# Autodesk Inventor assembly: Mud Kitchen 2.0
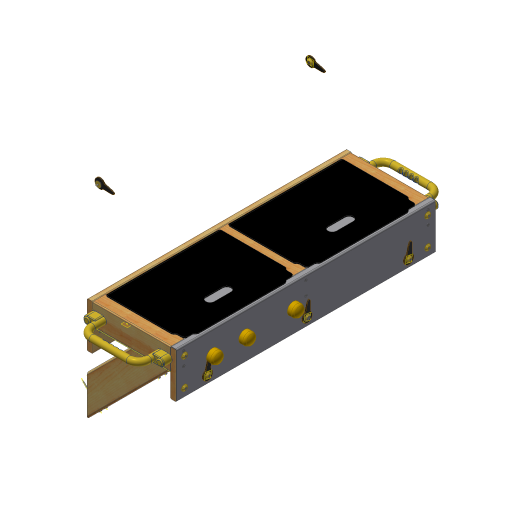
[picture p0: Inventor's stored thumbnail of the model, 512x512]
Saved by Autodesk Inventor 2024.3 (Build 283343000, 343)
## iProperties
Created: 2024-11-12
Part Number: Mud Kitchen 2.0
Document SubType Name: Assembly
Designer: l.hartouniyan
Assembly Measurements: /
Assembly Norm: /
Color: /
General Measurements: /
Packaging Manual: /
Packaging Method: /
Production Method: /
Tolerance: /
Weight: /
Author: l.hartouniyan
## Documents named in this file (14)
- Z:\Entwicklung\INVENTOR\4 Entwicklung\für 2024\24061_Mud kitchen 2.0\03_Product_development\01_3D_Construction\01_Assembly\Mud Kitchen 2.0.iam
- Z:\Entwicklung\INVENTOR\4 Entwicklung\für 2024\24061_Mud kitchen 2.0\03_Product_development\01_3D_Construction\03_Parts\Canvas\Tarp Mud Kitchen  2.0.ipt
- Z:\Entwicklung\INVENTOR\1 Teile\Holzteile\BK\Bauteile\BK-24.ipt
- Z:\Entwicklung\INVENTOR\1 Teile\Holzteile\B\Bauteile\B-80.ipt
- Z:\Entwicklung\INVENTOR\1 Teile\Holzteile\BG\Bauteile\BG-36.ipt
- Z:\Entwicklung\INVENTOR\1 Teile\Schrauben\Spannplattschrauben\Baugruppen Schrauben\5x20 inkl unterlegscheibe.iam
- Z:\Entwicklung\INVENTOR\1 Teile\Schrauben\Spannplattschrauben\Holzschraube-5x80mm.ipt
- Z:\Entwicklung\INVENTOR\1 Teile\Plastikteile\HDPE Platte\3mm\Baugruppe 3mm HDPE\Arrow Small 5x20mm washer.iam
- Z:\Entwicklung\INVENTOR\1 Teile\Schrauben\Spannplattschrauben\Holzschraube-4x50mm.ipt
- Z:\Entwicklung\INVENTOR\1 Teile\Plastikteile\GIANT\Deckel PRO gelb.ipt
- Z:\Entwicklung\INVENTOR\1 Teile\Plastikteile\GIANT\Kappe PRO gelb.ipt
- Z:\Entwicklung\INVENTOR\1 Teile\Plastikteile\Zubehör\Handgriff-gelb.ipt
- Z:\Entwicklung\INVENTOR\1 Teile\Plastikteile\Unterlegscheibe 18mm .ipt
- Z:\Entwicklung\INVENTOR\1 Teile\Plastikteile\HDPE Platte\3mm\oven deur 353 09.10 - gebogen.ipt
## Components (65 placed, 13 different names)
1. Tarp Mud Kitchen  2.0:1 — Flush:1, Flush:2, Flush:3, Flush:4, Flush:5, Flush:6, Flush:7, Mate:6, Tangent:22, Mate:7, Tangent:24, Mate:8, Tangent:26, Mate:9, Tangent:28, Mate:14, Mate:15, Tangent:57, Tangent:58, Tangent:59, Tangent:60, Mate:19, Mate:20, Mate:21, Tangent:94, Flush:56, Tangent:95, Flush:57, Mate:28
2. BK-24:1 — Flush:1, Flush:2, Flush:3, Flush:9, Mate:2, Flush:14, Mate:4, Flush:34, Tangent:49, Tangent:65, Tangent:67, Flush:46, Flush:47, Mate:18, Tangent:84, Tangent:85, Tangent:86, Tangent:87, Mate:26, Mate:30, Mate:31
3. BK-24:2 — Flush:4, Flush:5, Flush:6, Flush:8, Mate:1, Flush:10, Flush:15, Mate:5, Tangent:72, Tangent:73, Tangent:74, Tangent:75, Tangent:76, Tangent:77, Tangent:78, Tangent:79, Mate:27, Mate:33, Mate:34
4. BK-24:3 — Flush:7, Flush:8, Mate:1, Tangent:68, Tangent:69, Tangent:70, Tangent:71, Tangent:80, Tangent:81, Tangent:82, Tangent:83
5. B-80:1 — Flush:9, Flush:10, Mate:2, Tangent:21, Tangent:23, Tangent:25, Tangent:27, Tangent:50, Tangent:52, Tangent:54, Tangent:56, Flush:40, Tangent:64, Tangent:66, Tangent:88, Tangent:89, Tangent:90, Tangent:91, Tangent:92, Tangent:93
6. BG-36:1 — Flush:14, Mate:4, Tangent:45, Tangent:46, Tangent:47, Tangent:48, Tangent:51
7. BG-36:2 — Flush:15, Mate:5, Flush:30, Tangent:41, Tangent:42, Tangent:43, Tangent:44, Tangent:53, Tangent:55
8. 5x20 inkl unterlegscheibe:1 [sub-assembly] — Mate:6, Tangent:21, Tangent:22
9. 5x20 inkl unterlegscheibe:2 [sub-assembly] — Mate:7, Tangent:23, Tangent:24
10. 5x20 inkl unterlegscheibe:3 [sub-assembly] — Mate:8, Tangent:25, Tangent:26
11. 5x20 inkl unterlegscheibe:4 [sub-assembly] — Mate:9, Tangent:27, Tangent:28
12. Holzschraube-5x80mm:1 — Flush:30, Tangent:41, Tangent:42, Flush:31, Flush:32
13. Holzschraube-5x80mm:2 — Flush:31, Tangent:43, Tangent:44
14. Holzschraube-5x80mm:3 — Flush:32, Tangent:45, Tangent:46, Flush:33
15. Holzschraube-5x80mm:4 — Flush:33, Tangent:47, Tangent:48
16. Holzschraube-5x80mm:5 — Flush:34, Tangent:49, Tangent:50, Flush:35, Flush:36
17. Holzschraube-5x80mm:6 — Flush:35, Tangent:51, Tangent:52, Flush:37
18. Holzschraube-5x80mm:7 — Flush:36, Tangent:53, Tangent:54
19. Holzschraube-5x80mm:8 — Flush:37, Tangent:55, Tangent:56
20. oven deur 353 09.10 - gebogen:1 — Insert:5, Insert:6, Insert:18, Insert:19, Mate:29, Mate:30, Mate:31
21. oven deur 353 09.10 - gebogen:2 — Insert:3, Insert:4, Insert:20, Insert:21, Mate:32, Mate:33, Mate:34
22. 5x20 inkl unterlegscheibe:5 [sub-assembly] — Insert:20
23. 5x20 inkl unterlegscheibe:6 [sub-assembly] — Insert:21
24. 5x20 inkl unterlegscheibe:7 [sub-assembly] — Insert:3
25. 5x20 inkl unterlegscheibe:8 [sub-assembly] — Insert:18
26. 5x20 inkl unterlegscheibe:9 [sub-assembly] — Insert:4
27. 5x20 inkl unterlegscheibe:10 [sub-assembly] — Insert:6
28. 5x20 inkl unterlegscheibe:11 [sub-assembly] — Insert:19
29. 5x20 inkl unterlegscheibe:12 [sub-assembly] — Insert:5
30. Arrow Small 5x20mm washer:1 [sub-assembly] — Mate:15, Tangent:57, Tangent:58
31. Arrow Small 5x20mm washer:2 [sub-assembly] — Mate:14, Tangent:59, Tangent:60
32. Arrow Small 5x20mm washer:3 [sub-assembly] — Tangent:105, Flush:64, Tangent:106
33. Holzschraube-4x50mm:1 — Flush:40, Tangent:64, Tangent:65, Flush:41
34. Holzschraube-4x50mm:3 — Flush:41, Tangent:66, Tangent:67, Flush:42
35. Holzschraube-4x50mm:4 — Flush:42, Tangent:68, Tangent:69, Flush:43
36. Holzschraube-4x50mm:5 — Flush:43, Tangent:70, Tangent:71, Flush:44
37. Holzschraube-4x50mm:6 — Flush:44, Tangent:72, Tangent:73, Flush:45
38. Holzschraube-4x50mm:7 — Flush:45, Tangent:74, Tangent:75
39. B-80:2 — Flush:46, Flush:47, Mate:18, Flush:48, Flush:58, Tangent:96, Tangent:97, Flush:59, Tangent:98, Tangent:99, Flush:60, Tangent:100, Tangent:101, Flush:61, Tangent:102, Tangent:103, Tangent:105, Flush:64, Tangent:106, Flush:65, Tangent:107, Tangent:108, Mate:29, Mate:32
40. Holzschraube-4x50mm:8 — Flush:48, Tangent:76, Tangent:77, Flush:49
41. Holzschraube-4x50mm:9 — Flush:49, Tangent:78, Tangent:79, Flush:50
42. Holzschraube-4x50mm:10 — Flush:50, Tangent:80, Tangent:81, Flush:51
43. Holzschraube-4x50mm:11 — Flush:51, Tangent:82, Tangent:83, Flush:52
44. Holzschraube-4x50mm:12 — Flush:52, Tangent:84, Tangent:85, Flush:53
45. Holzschraube-4x50mm:13 — Flush:53, Tangent:86, Tangent:87
46. Deckel PRO gelb:1 — Insert:12
47. Kappe PRO gelb:1 — Tangent:88, Mate:19, Tangent:89, Insert:9, Insert:12, Insert:15
48. 5x20 inkl unterlegscheibe:13 [sub-assembly] — Insert:9
49. Kappe PRO gelb:2 — Tangent:90, Tangent:91, Mate:20, Insert:10, Insert:13, Insert:16
50. 5x20 inkl unterlegscheibe:14 [sub-assembly] — Insert:10
51. Kappe PRO gelb:3 — Tangent:92, Tangent:93, Mate:21, Insert:11, Insert:14, Insert:17
52. 5x20 inkl unterlegscheibe:15 [sub-assembly] — Insert:11
53. Deckel PRO gelb:2 — Insert:14
54. Deckel PRO gelb:3 — Insert:13
55. Arrow Small 5x20mm washer:4 [sub-assembly] — Flush:65, Tangent:107, Tangent:108
56. Handgriff-gelb:1 — Mate:26, Tangent:94, Flush:56
57. Handgriff-gelb:2 — Mate:27, Tangent:95, Flush:57
58. Holzschraube-4x50mm:14 — Flush:58, Tangent:96, Tangent:97
59. Holzschraube-4x50mm:15 — Flush:59, Tangent:98, Tangent:99
60. Holzschraube-4x50mm:16 — Flush:60, Tangent:100, Tangent:101
61. Holzschraube-4x50mm:17 — Flush:61, Tangent:102, Tangent:103
62. Unterlegscheibe 18mm :1 — Insert:15
63. Unterlegscheibe 18mm :2 — Insert:16
64. Unterlegscheibe 18mm :3 — Insert:17
65. Arrow Small 5x20mm washer:5 [sub-assembly] — Mate:28
## Relationships (154: Tangent 72, Flush 42, Mate 23, Insert 17)
- Flush:1: Tarp Mud Kitchen  2.0:1 ↔ BK-24:1
- Flush:2: Tarp Mud Kitchen  2.0:1 ↔ BK-24:1
- Flush:3: Tarp Mud Kitchen  2.0:1 ↔ BK-24:1
- Flush:4: Tarp Mud Kitchen  2.0:1 ↔ BK-24:2
- Flush:5: Tarp Mud Kitchen  2.0:1 ↔ BK-24:2
- Flush:6: Tarp Mud Kitchen  2.0:1 ↔ BK-24:2
- Flush:7: Tarp Mud Kitchen  2.0:1 ↔ BK-24:3
- Flush:8: BK-24:2 ↔ BK-24:3
- Mate:1 (334 mm): BK-24:2 ↔ BK-24:3
- Flush:9: BK-24:1 ↔ B-80:1
- Flush:10: BK-24:2 ↔ B-80:1
- Mate:2: BK-24:1 ↔ B-80:1
- Flush:14: BK-24:1 ↔ BG-36:1
- Mate:4: BK-24:1 ↔ BG-36:1
- Flush:15: BK-24:2 ↔ BG-36:2
- Mate:5: BK-24:2 ↔ BG-36:2
- Mate:6: Tarp Mud Kitchen  2.0:1 ↔ 5x20 inkl unterlegscheibe:1
- Tangent:21 (15 mm): B-80:1 ↔ 5x20 inkl unterlegscheibe:1
- Tangent:22 (15 mm): Tarp Mud Kitchen  2.0:1 ↔ 5x20 inkl unterlegscheibe:1
- Mate:7: Tarp Mud Kitchen  2.0:1 ↔ 5x20 inkl unterlegscheibe:2
- Tangent:23 (15 mm): B-80:1 ↔ 5x20 inkl unterlegscheibe:2
- Tangent:24 (15 mm): Tarp Mud Kitchen  2.0:1 ↔ 5x20 inkl unterlegscheibe:2
- Mate:8: Tarp Mud Kitchen  2.0:1 ↔ 5x20 inkl unterlegscheibe:3
- Tangent:25 (15 mm): B-80:1 ↔ 5x20 inkl unterlegscheibe:3
- Tangent:26 (15 mm): Tarp Mud Kitchen  2.0:1 ↔ 5x20 inkl unterlegscheibe:3
- Mate:9: Tarp Mud Kitchen  2.0:1 ↔ 5x20 inkl unterlegscheibe:4
- Tangent:27 (15 mm): B-80:1 ↔ 5x20 inkl unterlegscheibe:4
- Tangent:28 (15 mm): Tarp Mud Kitchen  2.0:1 ↔ 5x20 inkl unterlegscheibe:4
- Flush:30 (-1 mm): BG-36:2 ↔ Holzschraube-5x80mm:1
- Tangent:41 (25 mm): BG-36:2 ↔ Holzschraube-5x80mm:1
- Tangent:42 (20.25 mm): BG-36:2 ↔ Holzschraube-5x80mm:1
- Flush:31: Holzschraube-5x80mm:1 ↔ Holzschraube-5x80mm:2
- Tangent:43 (20.25 mm): BG-36:2 ↔ Holzschraube-5x80mm:2
- Tangent:44 (50 mm): BG-36:2 ↔ Holzschraube-5x80mm:2
- Flush:32: Holzschraube-5x80mm:1 ↔ Holzschraube-5x80mm:3
- Tangent:45 (20.25 mm): BG-36:1 ↔ Holzschraube-5x80mm:3
- Tangent:46 (25 mm): BG-36:1 ↔ Holzschraube-5x80mm:3
- Flush:33: Holzschraube-5x80mm:3 ↔ Holzschraube-5x80mm:4
- Tangent:47 (20.25 mm): BG-36:1 ↔ Holzschraube-5x80mm:4
- Tangent:48 (50 mm): BG-36:1 ↔ Holzschraube-5x80mm:4
- Flush:34 (-35 mm): BK-24:1 ↔ Holzschraube-5x80mm:5
- Tangent:49 (20.25 mm): BK-24:1 ↔ Holzschraube-5x80mm:5
- Tangent:50 (-40 mm): B-80:1 ↔ Holzschraube-5x80mm:5
- Flush:35 (-20.5 mm): Holzschraube-5x80mm:5 ↔ Holzschraube-5x80mm:6
- Tangent:51 (20.25 mm): BG-36:1 ↔ Holzschraube-5x80mm:6
- Tangent:52 (-60 mm): B-80:1 ↔ Holzschraube-5x80mm:6
- Flush:36: Holzschraube-5x80mm:5 ↔ Holzschraube-5x80mm:7
- Tangent:53 (20.25 mm): BG-36:2 ↔ Holzschraube-5x80mm:7
- Tangent:54 (-40 mm): B-80:1 ↔ Holzschraube-5x80mm:7
- Flush:37: Holzschraube-5x80mm:6 ↔ Holzschraube-5x80mm:8
- Tangent:55 (20.25 mm): BG-36:2 ↔ Holzschraube-5x80mm:8
- Tangent:56 (-60 mm): B-80:1 ↔ Holzschraube-5x80mm:8
- Insert:3: oven deur 353 09.10 - gebogen:2 ↔ 5x20 inkl unterlegscheibe:7
- Insert:4: oven deur 353 09.10 - gebogen:2 ↔ 5x20 inkl unterlegscheibe:9
- Insert:5: oven deur 353 09.10 - gebogen:1 ↔ 5x20 inkl unterlegscheibe:12
- Insert:6: oven deur 353 09.10 - gebogen:1 ↔ 5x20 inkl unterlegscheibe:10
- Mate:14: Tarp Mud Kitchen  2.0:1 ↔ Arrow Small 5x20mm washer:2
- Mate:15: Tarp Mud Kitchen  2.0:1 ↔ Arrow Small 5x20mm washer:1
- Tangent:57 (80 mm): Tarp Mud Kitchen  2.0:1 ↔ Arrow Small 5x20mm washer:1
- Tangent:58 (20 mm): Tarp Mud Kitchen  2.0:1 ↔ Arrow Small 5x20mm washer:1
- Tangent:59 (80 mm): Tarp Mud Kitchen  2.0:1 ↔ Arrow Small 5x20mm washer:2
- Tangent:60 (20 mm): Tarp Mud Kitchen  2.0:1 ↔ Arrow Small 5x20mm washer:2
- Flush:40 (-1 mm): B-80:1 ↔ Holzschraube-4x50mm:1
- Tangent:64 (20.5 mm): B-80:1 ↔ Holzschraube-4x50mm:1
- Tangent:65 (12 mm): BK-24:1 ↔ Holzschraube-4x50mm:1
- Flush:41: Holzschraube-4x50mm:1 ↔ Holzschraube-4x50mm:3
- Tangent:66 (20.5 mm): B-80:1 ↔ Holzschraube-4x50mm:3
- Tangent:67 (12 mm): BK-24:1 ↔ Holzschraube-4x50mm:3
- Flush:42: Holzschraube-4x50mm:3 ↔ Holzschraube-4x50mm:4
- Tangent:68 (20.5 mm): BK-24:3 ↔ Holzschraube-4x50mm:4
- Tangent:69 (12 mm): BK-24:3 ↔ Holzschraube-4x50mm:4
- Flush:43: Holzschraube-4x50mm:4 ↔ Holzschraube-4x50mm:5
- Tangent:70 (20.5 mm): BK-24:3 ↔ Holzschraube-4x50mm:5
- Tangent:71 (12 mm): BK-24:3 ↔ Holzschraube-4x50mm:5
- Flush:44: Holzschraube-4x50mm:5 ↔ Holzschraube-4x50mm:6
- Tangent:72 (20.5 mm): BK-24:2 ↔ Holzschraube-4x50mm:6
- Tangent:73 (12 mm): BK-24:2 ↔ Holzschraube-4x50mm:6
- Flush:45: Holzschraube-4x50mm:6 ↔ Holzschraube-4x50mm:7
- Tangent:74 (20.5 mm): BK-24:2 ↔ Holzschraube-4x50mm:7
- Tangent:75 (12 mm): BK-24:2 ↔ Holzschraube-4x50mm:7
- Flush:46: BK-24:1 ↔ B-80:2
- Flush:47: BK-24:1 ↔ B-80:2
- Mate:18: BK-24:1 ↔ B-80:2
- Flush:48 (-1 mm): B-80:2 ↔ Holzschraube-4x50mm:8
- Tangent:76 (20.5 mm): BK-24:2 ↔ Holzschraube-4x50mm:8
- Tangent:77 (12 mm): BK-24:2 ↔ Holzschraube-4x50mm:8
- Flush:49: Holzschraube-4x50mm:8 ↔ Holzschraube-4x50mm:9
- Tangent:78 (20.5 mm): BK-24:2 ↔ Holzschraube-4x50mm:9
- Tangent:79 (12 mm): BK-24:2 ↔ Holzschraube-4x50mm:9
- Flush:50: Holzschraube-4x50mm:9 ↔ Holzschraube-4x50mm:10
- Tangent:80 (20.5 mm): BK-24:3 ↔ Holzschraube-4x50mm:10
- Tangent:81 (12 mm): BK-24:3 ↔ Holzschraube-4x50mm:10
- Flush:51: Holzschraube-4x50mm:10 ↔ Holzschraube-4x50mm:11
- Tangent:82 (20.5 mm): BK-24:3 ↔ Holzschraube-4x50mm:11
- Tangent:83 (12 mm): BK-24:3 ↔ Holzschraube-4x50mm:11
- Flush:52: Holzschraube-4x50mm:11 ↔ Holzschraube-4x50mm:12
- Tangent:84 (20.5 mm): BK-24:1 ↔ Holzschraube-4x50mm:12
- Tangent:85 (12 mm): BK-24:1 ↔ Holzschraube-4x50mm:12
- Flush:53: Holzschraube-4x50mm:12 ↔ Holzschraube-4x50mm:13
- Tangent:86 (20.5 mm): BK-24:1 ↔ Holzschraube-4x50mm:13
- Tangent:87 (12 mm): BK-24:1 ↔ Holzschraube-4x50mm:13
- Tangent:88 (100 mm): B-80:1 ↔ Kappe PRO gelb:1
- Mate:19 (4.5 mm): Tarp Mud Kitchen  2.0:1 ↔ Kappe PRO gelb:1
- Tangent:89 (70 mm): B-80:1 ↔ Kappe PRO gelb:1
- Insert:9: Kappe PRO gelb:1 ↔ 5x20 inkl unterlegscheibe:13
- Tangent:90 (200 mm): B-80:1 ↔ Kappe PRO gelb:2
- Tangent:91 (70 mm): B-80:1 ↔ Kappe PRO gelb:2
- Mate:20 (4.5 mm): Tarp Mud Kitchen  2.0:1 ↔ Kappe PRO gelb:2
- Insert:10: Kappe PRO gelb:2 ↔ 5x20 inkl unterlegscheibe:14
- Tangent:92 (70 mm): B-80:1 ↔ Kappe PRO gelb:3
- Tangent:93 (350 mm): B-80:1 ↔ Kappe PRO gelb:3
- Mate:21 (4.5 mm): Tarp Mud Kitchen  2.0:1 ↔ Kappe PRO gelb:3
- Insert:11: Kappe PRO gelb:3 ↔ 5x20 inkl unterlegscheibe:15
- Insert:12: Deckel PRO gelb:1 ↔ Kappe PRO gelb:1
- Insert:13: Kappe PRO gelb:2 ↔ Deckel PRO gelb:3
- Insert:14: Kappe PRO gelb:3 ↔ Deckel PRO gelb:2
- Mate:26: BK-24:1 ↔ Handgriff-gelb:1
- Tangent:94 (-5 mm): Tarp Mud Kitchen  2.0:1 ↔ Handgriff-gelb:1
- Flush:56 (21.5 mm): Tarp Mud Kitchen  2.0:1 ↔ Handgriff-gelb:1
- Mate:27: BK-24:2 ↔ Handgriff-gelb:2
- Tangent:95 (-5 mm): Tarp Mud Kitchen  2.0:1 ↔ Handgriff-gelb:2
- Flush:57 (21.5 mm): Tarp Mud Kitchen  2.0:1 ↔ Handgriff-gelb:2
- Flush:58 (-1 mm): B-80:2 ↔ Holzschraube-4x50mm:14
- Tangent:96 (20.5 mm): B-80:2 ↔ Holzschraube-4x50mm:14
- Tangent:97 (23.5 mm): B-80:2 ↔ Holzschraube-4x50mm:14
- Flush:59 (-1 mm): B-80:2 ↔ Holzschraube-4x50mm:15
- Tangent:98 (20.5 mm): B-80:2 ↔ Holzschraube-4x50mm:15
- Tangent:99 (48.5 mm): B-80:2 ↔ Holzschraube-4x50mm:15
- Flush:60 (-1 mm): B-80:2 ↔ Holzschraube-4x50mm:16
- Tangent:100 (20.5 mm): B-80:2 ↔ Holzschraube-4x50mm:16
- Tangent:101 (23.5 mm): B-80:2 ↔ Holzschraube-4x50mm:16
- Flush:61 (-1 mm): B-80:2 ↔ Holzschraube-4x50mm:17
- Tangent:102 (20.5 mm): B-80:2 ↔ Holzschraube-4x50mm:17
- Tangent:103 (48.5 mm): B-80:2 ↔ Holzschraube-4x50mm:17
- Tangent:105 (245 mm): Arrow Small 5x20mm washer:3 ↔ B-80:2
- Flush:64 (68 mm): Arrow Small 5x20mm washer:3 ↔ B-80:2
- Tangent:106 (25 mm): Arrow Small 5x20mm washer:3 ↔ B-80:2
- Flush:65 (68 mm): B-80:2 ↔ Arrow Small 5x20mm washer:4
- Tangent:107 (245 mm): B-80:2 ↔ Arrow Small 5x20mm washer:4
- Tangent:108 (25 mm): B-80:2 ↔ Arrow Small 5x20mm washer:4
- Insert:15: Kappe PRO gelb:1 ↔ Unterlegscheibe 18mm :1
- Insert:16: Kappe PRO gelb:2 ↔ Unterlegscheibe 18mm :2
- Insert:17: Kappe PRO gelb:3 ↔ Unterlegscheibe 18mm :3
- Mate:28: Tarp Mud Kitchen  2.0:1 ↔ Arrow Small 5x20mm washer:5
- Insert:18: oven deur 353 09.10 - gebogen:1 ↔ 5x20 inkl unterlegscheibe:8
- Insert:19: oven deur 353 09.10 - gebogen:1 ↔ 5x20 inkl unterlegscheibe:11
- Mate:29: oven deur 353 09.10 - gebogen:1 ↔ B-80:2
- Mate:30: BK-24:1 ↔ oven deur 353 09.10 - gebogen:1
- Mate:31 (-9.5 mm): BK-24:1 ↔ oven deur 353 09.10 - gebogen:1
- Insert:20: oven deur 353 09.10 - gebogen:2 ↔ 5x20 inkl unterlegscheibe:5
- Insert:21: oven deur 353 09.10 - gebogen:2 ↔ 5x20 inkl unterlegscheibe:6
- Mate:32: oven deur 353 09.10 - gebogen:2 ↔ B-80:2
- Mate:33: BK-24:2 ↔ oven deur 353 09.10 - gebogen:2
- Mate:34 (-9.5 mm): BK-24:2 ↔ oven deur 353 09.10 - gebogen:2
